# Autodesk Inventor assembly: assembly_camera_mount_manual
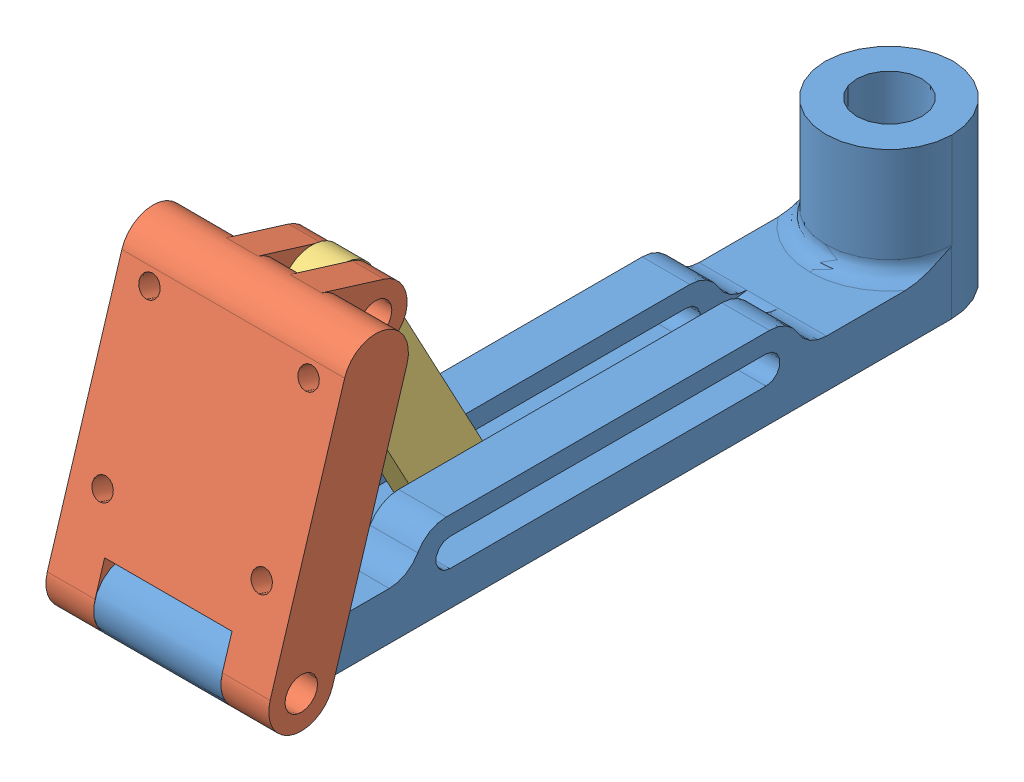
[picture p0: shaded view drawn from the shape stored in the file]
Saved by Autodesk Inventor 2021 (Build 250183000, 183)
## iProperties
Created: 2020-12-29
Part Number: assembly_camera_mount_manual
Document SubType Name: Assembly
Designer: Tomasz
Author: Tomasz
## Documents named in this file (4)
- D:\SynologyDrive\tcodev\tco-cad\mount_camera_manual\mount_camera_manual.iam
- D:\SynologyDrive\tcodev\tco-cad\mount_camera_manual\base.ipt
- D:\SynologyDrive\tcodev\tco-cad\mount_camera_manual\camera_arm.ipt
- D:\SynologyDrive\tcodev\tco-cad\mount_camera_manual\config_arm.ipt
## Components (3 placed, 3 different names)
1. base:1 — Mate:1, Mate:2, Tangent:1
2. camera_arm:1 — Mate:1, Mate:2, Mate:3, Mate:4
3. config_arm:1 — Mate:3, Mate:4, Tangent:1
## Relationships (5: Mate 4, Tangent 1)
- Mate:1: base:1 ↔ camera_arm:1
- Mate:2: base:1 ↔ camera_arm:1
- Mate:3: camera_arm:1 ↔ config_arm:1
- Mate:4: camera_arm:1 ↔ config_arm:1
- Tangent:1: base:1 ↔ config_arm:1
